# Autodesk Inventor assembly: element_newFeed
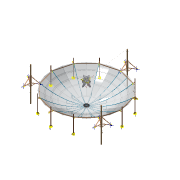
[picture p0: Inventor's stored thumbnail of the model, 180x180]
Saved by Autodesk Inventor 2017 (Build 210142000, 142)
## iProperties
Created: 2013-12-02
Part Number: element_newFeed
Document SubType Name: Assembly
Designer: Dave
Author: Dave
## Documents named in this file (30)
- C:\Users\Kathryn Rosie\Google Drive\HERA\hera-cad-0\element_newFeed.iam
- C:\Users\Kathryn Rosie\Google Drive\HERA\hera-cad-0\plat.ipt
- C:\Users\Kathryn Rosie\Google Drive\HERA\hera-cad-0\hub\hub.iam
- C:\Users\Kathryn Rosie\Google Drive\HERA\hera-cad-0\support\pole\poleAssembly.iam
- C:\Users\Kathryn Rosie\Google Drive\HERA\hera-cad-0\support\post\postAssembly.iam
- C:\Users\Kathryn Rosie\Google Drive\HERA\hera-cad-0\surface\sparFull.ipt
- C:\Users\Kathryn Rosie\Google Drive\HERA\hera-cad-0\support\sparAssembly.iam
- C:\Users\Kathryn Rosie\Google Drive\HERA\hera-cad-0\surface\crossAssembly_SA.iam
- C:\Users\Kathryn Rosie\Google Drive\HERA\hera-cad-0\surface\sparIntermediate.ipt
- C:\Users\Kathryn Rosie\Google Drive\HERA\hera-cad-0\surface\panels\panelA.ipt
- C:\Users\Kathryn Rosie\Google Drive\HERA\hera-cad-0\surface\panels\panelB.ipt
- C:\Users\Kathryn Rosie\Google Drive\HERA\hera-cad-0\surface\panels\panelC.ipt
- C:\Users\Kathryn Rosie\Google Drive\HERA\hera-cad-0\surface\panels\panelD.ipt
- C:\Users\Kathryn Rosie\Google Drive\HERA\hera-cad-0\surface\panels\panelE.ipt
- C:\Users\Kathryn Rosie\Google Drive\HERA\hera-cad-0\support\rimAssembly.iam
- C:\Users\Kathryn Rosie\Google Drive\HERA\hera-cad-0\support\kevlarFeed.ipt
- C:\Users\Kathryn Rosie\Google Drive\HERA\hera-cad-0\surface\screenInt.ipt
- C:\Users\Kathryn Rosie\Google Drive\HERA\hera-cad-0\surface\panels\panelBdoor.ipt
- C:\Users\Kathryn Rosie\Google Drive\HERA\hera-cad-0\jigs\totalStation.ipt
- C:\Users\Kathryn Rosie\Google Drive\HERA\hera-cad-0\jigs\vertex.ipt
- C:\Users\Kathryn Rosie\Google Drive\HERA\hera-cad-0\support\post\postStandSupport.iam
- C:\Users\Kathryn Rosie\Google Drive\HERA\hera-cad-0\jigs\centering.iam
- C:\Users\Kathryn Rosie\Google Drive\HERA\hera-cad-0\support\overlapStrip1.ipt
- C:\Users\Kathryn Rosie\Google Drive\HERA\hera-cad-0\support\overlapStrip2.ipt
- C:\Users\Kathryn Rosie\Google Drive\HERA\hera-cad-0\support\overlapStrip3.ipt
- C:\Users\Kathryn Rosie\Google Drive\HERA\hera-cad-0\surface\joinerBracket.ipt
- C:\Users\Kathryn Rosie\Google Drive\HERA\hera-cad-0\jigs\bridge.iam
- C:\Users\Kathryn Rosie\Google Drive\HERA\hera-cad-0\jigs\centerSpike.ipt
- C:\Users\Kathryn Rosie\Google Drive\HERA\hera-cad-0\smallParts\nail_20d.ipt
- C:\Users\Kathryn Rosie\Google Drive\HERA\hera-cad-0\feed\Feed\c7697-la-015_v0-7.iam
## Components (278 placed, 30 different names)
1. plat:1 — Insert:2, Angle:1, Angle:2, Angle:3, Angle:4, Mate:25
2. vertex:1 — Insert:19, Insert:20
3. hub:1 [sub-assembly] — Angle:5, Insert:19, Insert:23, Angle:14, Insert:30, Angle:16, Insert:33, Angle:22, Angle:23, Flush:2, Mate:26
4. panelBdoor:1
5. totalStation:1 — Insert:20
6. centeringjig:1 [sub-assembly] — Insert:21
7. kevlarFeedLine:1
8. c7697-la-015_v0-7:1 [sub-assembly] — Angle:23, Flush:2, Mate:26, Angle:24
9. bridge:1 [sub-assembly] — Mate:25
10. centerSpike:1 — Insert:33, Angle:22
11. sparIntermediate:1 — Insert:15, Angle:20
12. crossAssembly_SA:1 [sub-assembly] — Insert:15, Insert:29, Angle:15, Angle:20
13. panelA:1
14. panelA:2
15. panelA:3
16. panelA:4
17. panelA:5
18. panelA:6
19. panelA:7
20. panelA:8
21. panelA:9
22. panelA:10
23. panelA:11
24. panelA:12
25. panelB:1
26. panelB:2
27. panelB:3
28. panelB:4
29. panelB:5
30. panelB:6
31. panelB:7
32. panelB:8
33. panelB:9
34. panelB:10
35. panelB:11
36. panelB:12
37. panelB:13
38. panelB:14
39. panelB:15
40. panelB:16
41. panelB:17
42. panelB:18
43. panelB:19
44. panelB:20
45. panelB:21
46. panelB:22
47. panelB:23
48. panelC:1
49. panelD:1
50. panelE:1
51. panelC:2
52. panelD:2
53. panelE:2
54. panelC:3
55. panelD:3
56. panelE:3
57. panelC:4
58. panelD:4
59. panelE:4
60. panelC:5
61. panelD:5
62. panelE:5
63. panelC:6
64. panelD:6
65. panelE:6
66. panelC:7
67. panelD:7
68. panelE:7
69. panelC:8
70. panelD:8
71. panelE:8
72. panelC:9
73. panelD:9
74. panelE:9
75. panelC:10
76. panelD:10
77. panelE:10
78. panelC:11
79. panelD:11
80. panelE:11
81. panelC:12
82. panelD:12
83. panelE:12
84. panelC:13
85. panelD:13
86. panelE:13
87. panelC:14
88. panelD:14
89. panelE:14
90. panelC:15
91. panelD:15
92. panelE:15
93. panelC:16
94. panelD:16
95. panelE:16
96. panelC:17
97. panelD:17
98. panelE:17
99. panelC:18
100. panelD:18
101. panelE:18
102. panelC:19
103. panelD:19
104. panelE:19
105. panelC:20
106. panelD:20
107. panelE:20
108. panelC:21
109. panelD:21
110. panelE:21
111. panelC:22
112. panelD:22
113. panelE:22
114. panelC:23
115. panelD:23
116. panelE:23
117. panelC:24
118. panelD:24
119. panelE:24
120. screenInt:1
121. screenInt:2
122. screenInt:3
123. screenInt:4
124. screenInt:5
125. screenInt:6
126. screenInt:7
127. screenInt:8
128. screenInt:9
129. screenInt:10
130. screenInt:11
131. screenInt:12
132. poleAssembly:1 [sub-assembly] — Insert:2, Angle:1, Insert:21, Mate:22, Mate:23, Mate:24
133. postAssembly:1 [sub-assembly] — Angle:4
134. postStandSupport:1 [sub-assembly] — Mate:20, Flush:1, Mate:21
135. postAssembly:2 [sub-assembly] — Angle:3, Mate:20, Flush:1, Mate:21
136. postAssembly:3 [sub-assembly] — Angle:2
137. poleAssembly:2 [sub-assembly]
138. postAssembly:4 [sub-assembly]
139. postStandSupport:2 [sub-assembly]
140. postAssembly:5 [sub-assembly]
141. postAssembly:6 [sub-assembly]
142. poleAssembly:3 [sub-assembly]
143. postAssembly:7 [sub-assembly]
144. postStandSupport:3 [sub-assembly]
145. postAssembly:8 [sub-assembly]
146. postAssembly:9 [sub-assembly]
147. rimAssembly:1 [sub-assembly] — Mate:22, Mate:23, Mate:24
148. rimAssembly:2 [sub-assembly]
149. rimAssembly:3 [sub-assembly]
150. rimAssembly:4 [sub-assembly]
151. rimAssembly:5 [sub-assembly]
152. rimAssembly:6 [sub-assembly]
153. rimAssembly:7 [sub-assembly]
154. rimAssembly:8 [sub-assembly]
155. rimAssembly:9 [sub-assembly]
156. rimAssembly:10 [sub-assembly]
157. rimAssembly:11 [sub-assembly]
158. rimAssembly:12 [sub-assembly]
159. sparFull:1 — Insert:23, Insert:26, Insert:27, Insert:28, Angle:14, Insert:29, Angle:15, Angle:17, Angle:18, Angle:19
160. supportSparAssembly:1 [sub-assembly] — Angle:5, Insert:30, Angle:16
161. sparFull:2
162. sparAssembly:2 [sub-assembly]
163. sparFull:3
164. sparAssembly:3 [sub-assembly]
165. sparFull:4
166. sparAssembly:4 [sub-assembly]
167. sparFull:5
168. sparAssembly:5 [sub-assembly]
169. sparFull:6
170. sparAssembly:6 [sub-assembly]
171. sparFull:7
172. sparAssembly:7 [sub-assembly]
173. sparFull:8
174. sparAssembly:8 [sub-assembly]
175. sparFull:9
176. sparAssembly:9 [sub-assembly]
177. sparFull:10
178. sparAssembly:10 [sub-assembly]
179. sparFull:11
180. sparAssembly:11 [sub-assembly]
181. sparFull:12
182. sparAssembly:12 [sub-assembly]
183. nail_20d:1
184. nail_20d:2
185. nail_20d:3
186. nail_20d:4
187. nail_20d:5
188. nail_20d:6
189. nail_20d:7
190. nail_20d:8
191. nail_20d:9
192. nail_20d:10
193. nail_20d:11
194. nail_20d:12
195. overlapStrip3:1 — Insert:28, Angle:19
196. overlapStrip2:1 — Insert:27, Angle:18
197. overlapStrip1:1 — Insert:26, Angle:17
198. overlapStrip3:2
199. overlapStrip2:2
200. overlapStrip1:2
201. overlapStrip3:3
202. overlapStrip2:3
203. overlapStrip1:3
204. overlapStrip3:4
205. overlapStrip2:4
206. overlapStrip1:4
207. overlapStrip3:5
208. overlapStrip2:5
209. overlapStrip1:5
210. overlapStrip3:6
211. overlapStrip2:6
212. overlapStrip1:6
213. overlapStrip3:7
214. overlapStrip2:7
215. overlapStrip1:7
216. overlapStrip3:8
217. overlapStrip2:8
218. overlapStrip1:8
219. overlapStrip3:9
220. overlapStrip2:9
221. overlapStrip1:9
222. overlapStrip3:10
223. overlapStrip2:10
224. overlapStrip1:10
225. overlapStrip3:11
226. overlapStrip2:11
227. overlapStrip1:11
228. overlapStrip3:12
229. overlapStrip2:12
230. overlapStrip1:12
231. overlapStrip3:13
232. overlapStrip2:13
233. overlapStrip1:13
234. overlapStrip3:14
235. overlapStrip2:14
236. overlapStrip1:14
237. overlapStrip3:15
238. overlapStrip2:15
239. overlapStrip1:15
240. overlapStrip3:16
241. overlapStrip2:16
242. overlapStrip1:16
243. overlapStrip3:17
244. overlapStrip2:17
245. overlapStrip1:17
246. overlapStrip3:18
247. overlapStrip2:18
248. overlapStrip1:18
249. overlapStrip3:19
250. overlapStrip2:19
251. overlapStrip1:19
252. overlapStrip3:20
253. overlapStrip2:20
254. overlapStrip1:20
255. overlapStrip3:21
256. overlapStrip2:21
257. overlapStrip1:21
258. overlapStrip3:22
259. overlapStrip2:22
260. overlapStrip1:22
261. overlapStrip3:23
262. overlapStrip2:23
263. overlapStrip1:23
264. overlapStrip3:24
265. overlapStrip2:24
266. overlapStrip1:24
267. joinerBracket:1
268. joinerBracket:2
269. joinerBracket:3
270. joinerBracket:4
271. joinerBracket:5
272. joinerBracket:6
273. joinerBracket:7
274. joinerBracket:8
275. joinerBracket:9
276. joinerBracket:10
277. joinerBracket:11
278. joinerBracket:12
## Component patterns: panelA (12 elements), panelB (23 elements), panelC-E (24 elements), screen (12 elements), polesPosts (3 elements), rim (12 elements), fullSpar (12 elements), pins (12 elements), overlapStrips (24 elements), sparJoiner (12 elements)
## Relationships (36: Angle 15, Insert 12, Mate 7, Flush 2)
- Insert:2 (-1000 mm): plat:1 ↔ poleAssembly:1
- Angle:1 (90 deg): plat:1 ↔ poleAssembly:1
- Angle:2 (180 deg): plat:1 ↔ postAssembly:3
- Angle:3 (210 deg): plat:1 ↔ postAssembly:2
- Angle:4 (150 deg): plat:1 ↔ postAssembly:1
- Angle:5 (180 deg): hub:1 ↔ supportSparAssembly:1
- Insert:15 (-25.4 mm): sparIntermediate:1 ↔ crossAssembly_SA:1
- Insert:19 (82 mm): vertex:1 ↔ hub:1
- Insert:20 (-1524 mm): vertex:1 ↔ totalStation:1
- Mate:20: postStandSupport:1 ↔ postAssembly:2
- Flush:1: postStandSupport:1 ↔ postAssembly:2
- Mate:21 (1562.1 mm): postStandSupport:1 ↔ postAssembly:2
- Insert:21: centeringjig:1 ↔ poleAssembly:1
- Insert:23 (-314.5 mm): hub:1 ↔ sparFull:1
- Insert:26 (-63 mm): sparFull:1 ↔ overlapStrip1:1
- Insert:27 (-63 mm): sparFull:1 ↔ overlapStrip2:1
- Insert:28 (-63 mm): sparFull:1 ↔ overlapStrip3:1
- Angle:14 (180 deg): hub:1 ↔ sparFull:1
- Insert:29 (1 mm): crossAssembly_SA:1 ↔ sparFull:1
- Angle:15 (15 deg): crossAssembly_SA:1 ↔ sparFull:1
- Insert:30 (-38 mm): hub:1 ↔ supportSparAssembly:1
- Angle:16 (180 deg): hub:1 ↔ supportSparAssembly:1
- Angle:17 (173.1 deg): sparFull:1 ↔ overlapStrip1:1
- Angle:18 (173.5 deg): sparFull:1 ↔ overlapStrip2:1
- Angle:19 (186.25 deg): sparFull:1 ↔ overlapStrip3:1
- Mate:22: poleAssembly:1 ↔ rimAssembly:1
- Mate:23: poleAssembly:1 ↔ rimAssembly:1
- Mate:24 (-61 mm): poleAssembly:1 ↔ rimAssembly:1
- Angle:20 (180 deg): sparIntermediate:1 ↔ crossAssembly_SA:1
- Mate:25: plat:1 ↔ bridge:1
- Insert:33 (304.8 mm): hub:1 ↔ centerSpike:1
- Angle:22 (0 deg): hub:1 ↔ centerSpike:1
- Angle:23 (0 deg): hub:1 ↔ c7697-la-015_v0-7:1
- Flush:2 (-4500 mm): hub:1 ↔ c7697-la-015_v0-7:1
- Mate:26: hub:1 ↔ c7697-la-015_v0-7:1
- Angle:24 (0 deg): c7697-la-015_v0-7:1
